# Autodesk Inventor assembly: Fixed Caster
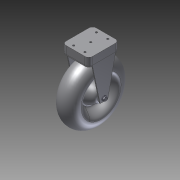
[picture p0: Inventor's stored thumbnail of the model, 180x180]
Saved by Autodesk Inventor 2012 (Build 160160000, 160)
## iProperties
Created: 2011-10-20
Part Number: Fixed Caster
Document SubType Name: Assembly
Designer: robotics
Author: robotics
## Documents named in this file (6)
- C:\Users\robotics\Dropbox\CAD Inventor\Preseason Projects\Cart Competition Cart\Team 2374\Fixed Caster.iam
- C:\Users\robotics\Dropbox\CAD Inventor\Preseason Projects\Cart Competition Cart\Team 2374\Caster2.ipt
- C:\Users\robotics\Dropbox\CAD Inventor\Preseason Projects\Cart Competition Cart\Team 2374\Wheel.ipt
- C:\Users\robotics\Dropbox\CAD Inventor\Preseason Projects\Cart Competition Cart\Team 2374\Spacer - .5 x .25.ipt
- C:\Users\robotics\Dropbox\CAD Inventor\Preseason Projects\Cart Competition Cart\Team 2374\Caster\Design Accelerator\Bolted Connection1.iam
- C:\Users\robotics\Dropbox\CAD Inventor\Preseason Projects\Cart Competition Cart\Team 2374\Fixed Extension.ipt
## Components (6 placed, 5 different names)
1. Caster2:1 — Mate:1, Mate:2, Mate:3, Mate:4, Mate:5, Mate:6, Mate:7, Mate:21, Mate:22, Flush:1, Flush:2, Mate:23
2. Wheel:1 — Mate:1, Mate:2, Mate:3
3. Spacer - .5 x .25:1 — Mate:4, Mate:5
4. Spacer - .5 x .25:2 — Mate:6, Mate:7
5. Bolted Connection:1 [sub-assembly] — Mate:21, Mate:22
6. Fixed Extension:1 — Flush:1, Flush:2, Mate:23
## Relationships (12: Mate 10, Flush 2)
- Mate:1 (6.35 mm): Caster2:1 ↔ Wheel:1
- Mate:2 (111.125 mm): Caster2:1 ↔ Wheel:1
- Mate:3 (-50.8 mm): Caster2:1 ↔ Wheel:1
- Mate:4: Caster2:1 ↔ Spacer - .5 x .25:1
- Mate:5: Caster2:1 ↔ Spacer - .5 x .25:1
- Mate:6: Caster2:1 ↔ Spacer - .5 x .25:2
- Mate:7: Caster2:1 ↔ Spacer - .5 x .25:2
- Mate:21: Caster2:1 ↔ Bolted Connection:1
- Mate:22: Caster2:1 ↔ Bolted Connection:1
- Flush:1: Caster2:1 ↔ Fixed Extension:1
- Flush:2: Caster2:1 ↔ Fixed Extension:1
- Mate:23: Caster2:1 ↔ Fixed Extension:1
